# Autodesk Inventor assembly: Fixture Assembly
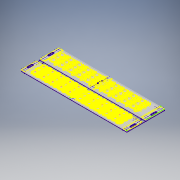
[picture p0: Inventor's stored thumbnail of the model, 180x180]
Saved by Autodesk Inventor 2018 (Build 220112000, 112)
## iProperties
Created: 2016-04-08
Part Number: Fixture Assembly
Document SubType Name: Assembly
Designer: Sam Clay
Author: Sam Clay
## Documents named in this file (6)
- Z:\enclosure\inventor\Fixture Assembly.iam
- Z:\enclosure\inventor\Fixture Base.ipt
- Z:\enclosure\inventor\Case Top Contour Fixture.ipt
- Z:\enclosure\inventor\Case Bottom Contour Fixture.ipt
- Z:\enclosure\inventor\Case Top Pocket Fixture.ipt
- Z:\enclosure\inventor\Case Bottom Pocket Fixture.ipt
## Components (121 placed, 5 different names)
1. Fixture Base:1 — Mate:27, Mate:28, Mate:35, Mate:36, Mate:38, Flush:1
2. Case Top Pocket Fixture:1 — Mate:34, Mate:35, Mate:36, Mate:39
3. Case Bottom Pocket Fixture:1 — Mate:34, Mate:38, Mate:39
4. Case Top Pocket Fixture:3
5. Case Bottom Pocket Fixture:2
6. Case Top Pocket Fixture:4
7. Case Bottom Pocket Fixture:3
8. Case Top Pocket Fixture:5
9. Case Bottom Pocket Fixture:4
10. Case Top Pocket Fixture:6
11. Case Bottom Pocket Fixture:5
12. Case Top Pocket Fixture:7
13. Case Bottom Pocket Fixture:6
14. Case Top Pocket Fixture:8
15. Case Bottom Pocket Fixture:7
16. Case Top Pocket Fixture:9
17. Case Bottom Pocket Fixture:8
18. Case Top Pocket Fixture:10
19. Case Bottom Pocket Fixture:9
20. Case Top Pocket Fixture:11
21. Case Bottom Pocket Fixture:10
22. Case Top Pocket Fixture:12
23. Case Bottom Pocket Fixture:11
24. Case Top Pocket Fixture:13
25. Case Bottom Pocket Fixture:12
26. Case Top Pocket Fixture:14
27. Case Bottom Pocket Fixture:13
28. Case Top Pocket Fixture:15
29. Case Bottom Pocket Fixture:14
30. Case Top Pocket Fixture:16
31. Case Bottom Pocket Fixture:15
32. Case Top Pocket Fixture:17
33. Case Bottom Pocket Fixture:16
34. Case Top Pocket Fixture:18
35. Case Bottom Pocket Fixture:17
36. Case Top Pocket Fixture:19
37. Case Bottom Pocket Fixture:18
38. Case Top Pocket Fixture:20
39. Case Bottom Pocket Fixture:19
40. Case Top Pocket Fixture:21
41. Case Bottom Pocket Fixture:20
42. Case Top Pocket Fixture:22
43. Case Bottom Pocket Fixture:21
44. Case Top Pocket Fixture:23
45. Case Bottom Pocket Fixture:22
46. Case Top Pocket Fixture:24
47. Case Bottom Pocket Fixture:23
48. Case Top Pocket Fixture:25
49. Case Bottom Pocket Fixture:24
50. Case Top Pocket Fixture:26
51. Case Bottom Pocket Fixture:25
52. Case Top Pocket Fixture:27
53. Case Bottom Pocket Fixture:26
54. Case Top Pocket Fixture:28
55. Case Bottom Pocket Fixture:27
56. Case Top Pocket Fixture:29
57. Case Bottom Pocket Fixture:28
58. Case Top Pocket Fixture:30
59. Case Bottom Pocket Fixture:29
60. Case Top Pocket Fixture:31
61. Case Bottom Pocket Fixture:30
62. Case Top Contour Fixture:1 — Mate:27, Mate:28, Mate:31, Mate:32
63. Case Bottom Contour Fixture:16 — Mate:31, Mate:32, Flush:1
64. Case Top Contour Fixture:2
65. Case Bottom Contour Fixture:17
66. Case Top Contour Fixture:3
67. Case Bottom Contour Fixture:18
68. Case Top Contour Fixture:4
69. Case Bottom Contour Fixture:19
70. Case Top Contour Fixture:5
71. Case Bottom Contour Fixture:20
72. Case Top Contour Fixture:6
73. Case Bottom Contour Fixture:21
74. Case Top Contour Fixture:7
75. Case Bottom Contour Fixture:22
76. Case Top Contour Fixture:8
77. Case Bottom Contour Fixture:23
78. Case Top Contour Fixture:9
79. Case Bottom Contour Fixture:24
80. Case Top Contour Fixture:11
81. Case Bottom Contour Fixture:25
82. Case Top Contour Fixture:12
83. Case Bottom Contour Fixture:26
84. Case Top Contour Fixture:13
85. Case Bottom Contour Fixture:27
86. Case Top Contour Fixture:14
87. Case Bottom Contour Fixture:28
88. Case Top Contour Fixture:15
89. Case Bottom Contour Fixture:29
90. Case Top Contour Fixture:16
91. Case Bottom Contour Fixture:30
92. Case Top Contour Fixture:17
93. Case Bottom Contour Fixture:31
94. Case Top Contour Fixture:18
95. Case Bottom Contour Fixture:32
96. Case Top Contour Fixture:19
97. Case Bottom Contour Fixture:33
98. Case Top Contour Fixture:20
99. Case Bottom Contour Fixture:34
100. Case Top Contour Fixture:21
101. Case Bottom Contour Fixture:35
102. Case Top Contour Fixture:22
103. Case Bottom Contour Fixture:36
104. Case Top Contour Fixture:23
105. Case Bottom Contour Fixture:37
106. Case Top Contour Fixture:24
107. Case Bottom Contour Fixture:38
108. Case Top Contour Fixture:25
109. Case Bottom Contour Fixture:39
110. Case Top Contour Fixture:26
111. Case Bottom Contour Fixture:40
112. Case Top Contour Fixture:27
113. Case Bottom Contour Fixture:41
114. Case Top Contour Fixture:28
115. Case Bottom Contour Fixture:42
116. Case Top Contour Fixture:29
117. Case Bottom Contour Fixture:43
118. Case Top Contour Fixture:30
119. Case Bottom Contour Fixture:44
120. Case Top Contour Fixture:31
121. Case Bottom Contour Fixture:45
## Component patterns: (2 elements), (2 elements), (15 elements, first: Case Top Pocket Fixture:1 + Case Bottom Pocket Fixture:1), Component Pattern 10:2 (15 elements), (15 elements, first: Case Top Contour Fixture:1 + Case Bottom Contour Fixture:16), Component Pattern 3:2 (15 elements)
## Relationships (10: Mate 9, Flush 1)
- Mate:27 (-19.05 mm): Fixture Base:1 ↔ Case Top Contour Fixture:1
- Mate:28 (-63.5 mm): Fixture Base:1 ↔ Case Top Contour Fixture:1
- Mate:31: Case Top Contour Fixture:1 ↔ Case Bottom Contour Fixture:16
- Mate:32 (6.604 mm): Case Top Contour Fixture:1 ↔ Case Bottom Contour Fixture:16
- Flush:1 (-16.51 mm): Fixture Base:1 ↔ Case Bottom Contour Fixture:16
- Mate:34: Case Top Pocket Fixture:1 ↔ Case Bottom Pocket Fixture:1
- Mate:35 (6.35 mm): Fixture Base:1 ↔ Case Top Pocket Fixture:1
- Mate:36 (1.27 mm): Fixture Base:1 ↔ Case Top Pocket Fixture:1
- Mate:38: Fixture Base:1 ↔ Case Bottom Pocket Fixture:1
- Mate:39 (6.604 mm): Case Top Pocket Fixture:1 ↔ Case Bottom Pocket Fixture:1
